# Autodesk Inventor assembly: Foot
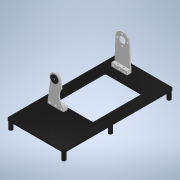
[picture p0: Inventor's stored thumbnail of the model, 180x180]
Saved by Autodesk Inventor 2020.4 (Build 244396000, 396)
## iProperties
Created: 2021-09-07
Part Number: Foot
Document SubType Name: Assembly
Designer: naoki
Mass: 68.6803 g
Surface Area: 351.037 cm^2
Volume: 41.2832 cm^3
Density: 1.66364 g/cm^3
Author: naoki
Title: Foot
## Documents named in this file (10)
- C:\Users\Masato\Desktop\OpenPlatform_ver3_0\LowerBody\Foot\foot.iam
- Foot.iam
- C:\Users\Masato\Desktop\OpenPlatform_ver3_0\LowerBody\Foot\sole.ipt
- C:\Users\Masato\Desktop\OpenPlatform_ver3_0\LowerBody\Foot\Foot_vertical_01.ipt
- C:\Users\Masato\Desktop\OpenPlatform_ver3_0\Ready_Made\ARU-313SMO.ipt
- C:\Users\Masato\Desktop\OpenPlatform_ver3_0\LowerBody\Foot\Foot_roll_vertical_02.ipt
- C:\Users\Masato\Desktop\OpenPlatform_ver3_0\LowerBody\Foot\Foot_roll_vertical_01.ipt
- C:\Users\Masato\Desktop\OpenPlatform_ver3_0\Ready_Made\80F-0603.ipt
- C:\Users\Masato\Desktop\OpenPlatform_ver3_0\Ready_Made\LFW-0815.ipt
- C:\Users\Masato\Desktop\OpenPlatform_ver3_0\Ready_Made\UUW-0312-10BH.ipt
## Components (14 placed, 8 different names)
1. sole:1 — 挿入:1, 挿入:2, 挿入:3, 挿入:4, 挿入:5, 挿入:6, 挿入:7, 挿入:8, 挿入:9, 挿入:10, メイト:1, メイト:2, メイト:3
2. Foot_vertical_01:1 — 挿入:1, 挿入:2, 挿入:11, 挿入:12, 挿入:13
3. Foot_vertical_01:2 — 挿入:3, 挿入:4, 挿入:14, 挿入:15
4. ARL-313SBE:1 — 挿入:10
5. ARL-313SBE:2 — 挿入:9
6. ARL-313SBE:3 — 挿入:8
7. ARL-313SBE:4 — 挿入:7
8. ARL-313SBE:5 — 挿入:6
9. ARL-313SBE:6 — 挿入:5
10. Foot_roll_vertical_02:1 — 挿入:14, 挿入:15
11. Foot_roll_vertical_01:1 — 挿入:11, 挿入:12, 挿入:13, 挿入:16, 挿入:17
12. 80F-0603:1 — 挿入:16
13. LFW-0815:1 — 挿入:17, 挿入:18
14. UUW-0312-10BH:1 — 挿入:18
## Relationships (21: Insert 18, Mate 3)
- 挿入:1 [Insert]: sole:1 ↔ Foot_vertical_01:1
- 挿入:2 [Insert]: sole:1 ↔ Foot_vertical_01:1
- 挿入:3 [Insert]: sole:1 ↔ Foot_vertical_01:2
- 挿入:4 [Insert]: sole:1 ↔ Foot_vertical_01:2
- 挿入:5 [Insert]: sole:1 ↔ ARL-313SBE:6
- 挿入:6 [Insert]: sole:1 ↔ ARL-313SBE:5
- 挿入:7 [Insert]: sole:1 ↔ ARL-313SBE:4
- 挿入:8 [Insert]: sole:1 ↔ ARL-313SBE:3
- 挿入:9 [Insert]: sole:1 ↔ ARL-313SBE:2
- 挿入:10 [Insert]: sole:1 ↔ ARL-313SBE:1
- 挿入:11 [Insert]: Foot_vertical_01:1 ↔ Foot_roll_vertical_01:1
- 挿入:12 [Insert]: Foot_vertical_01:1 ↔ Foot_roll_vertical_01:1
- 挿入:13 [Insert]: Foot_vertical_01:1 ↔ Foot_roll_vertical_01:1
- 挿入:14 [Insert]: Foot_vertical_01:2 ↔ Foot_roll_vertical_02:1
- 挿入:15 [Insert]: Foot_vertical_01:2 ↔ Foot_roll_vertical_02:1
- 挿入:16 [Insert]: Foot_roll_vertical_01:1 ↔ 80F-0603:1
- 挿入:17 [Insert]: Foot_roll_vertical_01:1 ↔ LFW-0815:1
- 挿入:18 [Insert]: LFW-0815:1 ↔ UUW-0312-10BH:1
- メイト:1 [Mate]: sole:1
- メイト:2 [Mate]: sole:1
- メイト:3 [Mate]: sole:1
